# Autodesk Inventor assembly: AmpFlow Motor & Gearbox
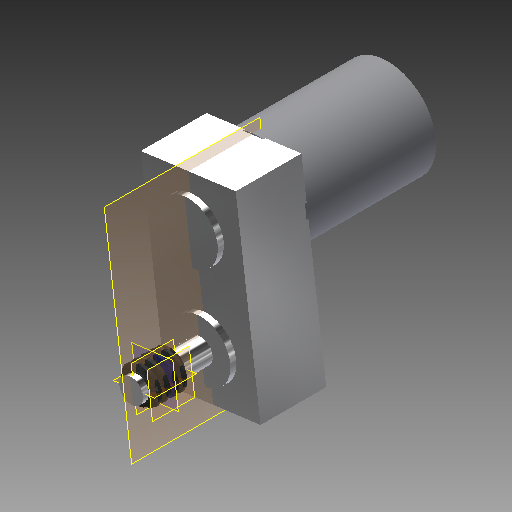
[picture p0: Inventor's stored thumbnail of the model, 512x512]
Saved by Autodesk Inventor 2019 (Build 230136000, 136)
## iProperties
Created: 2018-10-29
Part Number: AmpFlow Motor & Gearbox
Document SubType Name: Assembly
Designer: Alex Barnett
Mass: 2280.05 g
Surface Area: 966.42 cm^2
Volume: 1130.32 cm^3
Density: 2.01718 g/cm^3
Author: Alex Barnett
## Documents named in this file (4)
- C:\Users\Alex Barnett\Documents\Machine Design\PR2\CAD\AmpFlow Motor & Gearbox.iam
- C:\Users\Alex Barnett\Documents\Machine Design\PR2\CAD\Amplow A28-150 Motor.ipt
- C:\Users\Alex Barnett\Documents\Machine Design\PR2\CAD\A28-400-G Gearbox.ipt
- C:\Users\Alex Barnett\Documents\Machine Design\PR2\CAD\Worm 12P .5in. ID.ipt
## Components (3 placed, 3 different names)
1. Amplow A28-150 Motor:1 — Mate:1, Mate:2
2. A28-400-G Gearbox:1 — Mate:1, Mate:2, Mate:3, Flush:1, Flush:2
3. Worm 12P .5in. ID:1 — Mate:3, Flush:1, Flush:2
## Relationships (5: Mate 3, Flush 2)
- Mate:1: Amplow A28-150 Motor:1 ↔ A28-400-G Gearbox:1
- Mate:2: Amplow A28-150 Motor:1 ↔ A28-400-G Gearbox:1
- Mate:3: A28-400-G Gearbox:1 ↔ Worm 12P .5in. ID:1
- Flush:1 (-50.8 mm): A28-400-G Gearbox:1 ↔ Worm 12P .5in. ID:1
- Flush:2: A28-400-G Gearbox:1 ↔ Worm 12P .5in. ID:1
